# Autodesk Inventor assembly: Subsystem_1
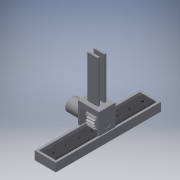
[picture p0: Inventor's stored thumbnail of the model, 180x180]
Saved by Autodesk Inventor 2019.4 (Build 234330000, 330)
## iProperties
Created: 2020-04-15
Part Number: Subsystem_1
Document SubType Name: Assembly
Designer: Niran
Author: Niran
## iProperties of the stored document S.motor.ipt
Created: 2020-04-14
Part Number: S.motor
Material: Generic
Document SubType Name: Modeling
Designer: Darugar
Density: 1 g/cm^3
Appearance: Default
Author: Darugar
Sending System: Autodesk Inventor 2020
## iProperties of the stored document S.hollow box.ipt
Created: 2020-04-13
Part Number: S.hollow box
Material: Generic
Document SubType Name: Modeling
Designer: Darugar
Density: 1 g/cm^3
Appearance: Default
Author: Darugar
Sending System: Autodesk Inventor 2020
## iProperties of the stored document S.rack.ipt
Created: 2020-04-14
Part Number: S.rack
Material: Generic
Document SubType Name: Modeling
Designer: Darugar
Density: 1 g/cm^3
Appearance: Default
Author: Darugar
Sending System: Autodesk Inventor 2020
## iProperties of the stored document S.Platform.ipt
Created: 2020-04-14
Part Number: S.Platform
Material: Generic
Document SubType Name: Modeling
Designer: Darugar
Density: 1 g/cm^3
Appearance: Default
Author: Darugar
Sending System: Autodesk Inventor 2020
## iProperties of the stored document S.gear.ipt
Created: 2020-04-14
Part Number: S.gear
Material: Generic
Document SubType Name: Modeling
Designer: Darugar
Density: 1 g/cm^3
Appearance: Default
Author: Darugar
Sending System: Autodesk Inventor 2020
## Documents named in this file (11)
- **C:\Users\Niran\Desktop\S.Carrom_bot\Subsystem_1.iam*LocalDocs*xLcir2i3dJi23ejcuSf5cnstxGa*S.motor.ipt
- **C:\Users\Niran\Desktop\S.Carrom_bot\Subsystem_1.iam*LocalDocs*xHt5motkgAg1kewgg2tsufwgnGg*S.hollow box.ipt
- **C:\Users\Niran\Desktop\S.Carrom_bot\Subsystem_1.iam*LocalDocs*x5nogo2nhHjxtulshHm4yuap04h*S.rack.ipt
- **C:\Users\Niran\Desktop\S.Carrom_bot\Subsystem_1.iam*LocalDocs*xI1ac5dbeIwp4uus51jjvtkad4f*S.Platform.ipt
- **C:\Users\Niran\Desktop\S.Carrom_bot\Subsystem_1.iam*LocalDocs*xUfgzfs1eU502u200I0wxzhccAh*S.gear.ipt
- C:\Users\Niran\Desktop\S.Carrom_bot\Subsystem_1.iam
- C:\Users\Niran\Desktop\S.Carrom_bot\S.rack.ipt
- C:\Users\Niran\Desktop\S.Carrom_bot\S.hollow box.ipt
- C:\Users\Niran\Desktop\S.Carrom_bot\S.Platform.ipt
- C:\Users\Niran\Desktop\S.Carrom_bot\S.motor.ipt
- C:\Users\Niran\Desktop\S.Carrom_bot\S.gear.ipt
## Components (5 placed, 5 different names)
1. S.rack:1 — Rotational:1
2. S.hollow box:1 — Rotational:1, Rotational:2
3. S.Platform:1 — Rotational:2, Rigid:1
4. S.motor:1 — Rigid:1, Rigid:2
5. S.gear:1 — Rigid:2
## Relationships (4: RevoluteJoint 2, WeldJoint 2)
- Rotational:1 [RevoluteJoint]: S.rack:1 ↔ S.hollow box:1
- Rotational:2 [RevoluteJoint]: S.hollow box:1 ↔ S.Platform:1
- Rigid:1 [WeldJoint] (-10 mm): S.Platform:1 ↔ S.motor:1
- Rigid:2 [WeldJoint] (20 mm): S.motor:1 ↔ S.gear:1
